# Autodesk Inventor assembly: AM14U3+Long+REV1-1
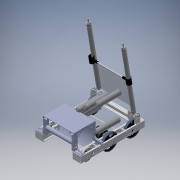
[picture p0: Inventor's stored thumbnail of the model, 180x180]
Saved by Autodesk Inventor 2016 (Build 200138000, 138)
## iProperties
Created: 2015-12-07
Part Number: AM14U3+Long+REV1-1
Description: STEP AP214
Document SubType Name: Assembly
Designer: Douglas
Sending System: SolidWorks 2014
Preprocessor: SwSTEP 2.0
Title: AM14U3 Long REV2.STEP
Revision Number: ANY
## Documents named in this file (7)
- D:\SkyDrive\GitHub\2016-Robot-CAD\Inventor\Chassis\AM14U3+Long+REV1-1.iam
- D:\SkyDrive\GitHub\2016-Robot-CAD\Inventor\PARTS\TMP.ipt
- D:\SkyDrive\GitHub\2016-Robot-CAD\Inventor\Lift.iam
- D:\SkyDrive\GitHub\2016-Robot-CAD\Inventor\Manipulator.iam
- D:\SkyDrive\GitHub\2016-Robot-CAD\Inventor\Chassis\Left Side.iam
- D:\SkyDrive\GitHub\2016-Robot-CAD\Inventor\Chassis\Right Side.iam
- D:\SkyDrive\GitHub\2016-Robot-CAD\Inventor\PARTS\Storage Tank\Storage-Tank-avt-pp-35.iam
## Components (15 placed, 6 different names)
1. TMP:1
2. Lift:1 [sub-assembly] — Mate:10, Mate:11
3. Manipulator:2 [sub-assembly] — Mate:5, Mate:8, Mate:9
4. Left Side:1 [sub-assembly] — Mate:1, Mate:2, Mate:4, Mate:5, Mate:6, Mate:7, Mate:9
5. Right Side:1 [sub-assembly] — Mate:1, Mate:2, Mate:3, Mate:4, Mate:6, Mate:7, Mate:8, Mate:10, Mate:11
6. Storage-Tank-avt-pp-35:1 [sub-assembly]
7. Storage-Tank-avt-pp-35:2 [sub-assembly]
8. Storage-Tank-avt-pp-35:3 [sub-assembly]
9. Storage-Tank-avt-pp-35:4 [sub-assembly]
10. Storage-Tank-avt-pp-35:5 [sub-assembly]
11. Storage-Tank-avt-pp-35:6 [sub-assembly]
12. Storage-Tank-avt-pp-35:7 [sub-assembly]
13. Storage-Tank-avt-pp-35:8 [sub-assembly]
14. Storage-Tank-avt-pp-35:9 [sub-assembly]
15. Storage-Tank-avt-pp-35:10 [sub-assembly]
## Relationships (11: Mate 11)
- Mate:1: Left Side:1 ↔ Right Side:1
- Mate:2: Left Side:1 ↔ Right Side:1
- Mate:3: Right Side:1
- Mate:4: Left Side:1 ↔ Right Side:1
- Mate:5: Manipulator:2 ↔ Left Side:1
- Mate:6: Left Side:1 ↔ Right Side:1
- Mate:7: Left Side:1 ↔ Right Side:1
- Mate:8: Manipulator:2 ↔ Right Side:1
- Mate:9: Manipulator:2 ↔ Left Side:1
- Mate:10: Lift:1 ↔ Right Side:1
- Mate:11: Lift:1 ↔ Right Side:1
